# Autodesk Inventor assembly: WinderAssembly
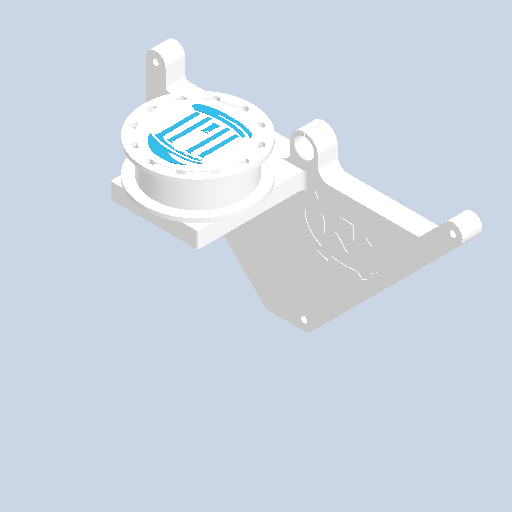
[picture p0: Inventor's stored thumbnail of the model, 512x512]
Saved by Autodesk Inventor 2022 (Build 260153000, 153)
## iProperties
Created: 2020-03-15
Part Number: WinderAssembly
Document SubType Name: Assembly
Designer: elmar
Author: elmar
## Documents named in this file (3)
- C:\repo\FourWireBraidingMachine\MetalCableBraider\WinderAssembly.iam
- C:\repo\FourWireBraidingMachine\MetalCableBraider\WinderSpool.ipt
- C:\repo\FourWireBraidingMachine\MetalCableBraider\WinderBracket.ipt
## Components (2 placed, 2 different names)
1. WinderSpool:1 — Insert:1
2. WinderBracket:1 — Insert:1
## Relationships (1: Insert 1)
- Insert:1 (1 mm): WinderSpool:1 ↔ WinderBracket:1
